# Autodesk Inventor assembly: Cangrejo-Sin-Reductores
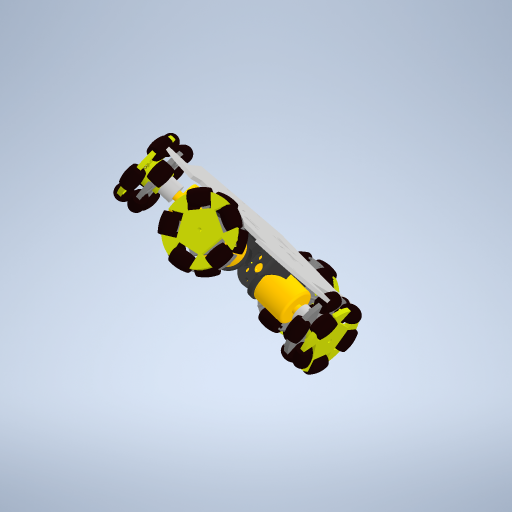
[picture p0: Inventor's stored thumbnail of the model, 512x512]
Saved by Autodesk Inventor 2024 (Build 280153000, 153)
## iProperties
Created: 2023-11-21
Part Number: Cangrejo-Sin-Reductores
Document SubType Name: Assembly
Designer: felip
Author: felip
## Documents named in this file (5)
- C:\Users\felip\Downloads\Gemelo Digital V2\Cangrejo-Sin-Reductores.iam
- C:\Users\felip\Downloads\Gemelo Digital V2\Motor-Soporte-Montaje.iam
- C:\Users\felip\Downloads\Gemelo Digital V2\OMNIWHEELV4.iam
- C:\Users\felip\Downloads\Gemelo Digital V2\Pseudo-SunGear.ipt
- C:\Users\felip\Downloads\Gemelo Digital V2\BaseV7.5.ipt
## Components (13 placed, 4 different names)
1. Motor-Soporte-Montaje:1 [sub-assembly] — Rotational:7, Rotational:22, Rotational:23
2. OMNIWHEELV4:1 [sub-assembly] — Rotational:14
3. Pseudo-SunGear:2 — Rotational:7, Rotational:17
4. Pseudo-SunGear:4 — Rotational:8, Rotational:14
5. Motor-Soporte-Montaje:2 [sub-assembly] — Rotational:8, Rotational:20, Rotational:21
6. OMNIWHEELV4:2 [sub-assembly] — Rotational:9
7. OMNIWHEELV4:4 [sub-assembly] — Rotational:17
8. Pseudo-SunGear:5 — Rotational:9
9. Motor-Soporte-Montaje:4 [sub-assembly] — Rotational:24, Rotational:25
10. OMNIWHEELV4:5 [sub-assembly]
11. Pseudo-SunGear:6
12. Motor-Soporte-Montaje:5 [sub-assembly] — Rotational:18, Rotational:19
13. BaseV7.5:1 — Rotational:18, Rotational:19, Rotational:20, Rotational:21, Rotational:22, Rotational:23, Rotational:24, Rotational:25
## Relationships (16: RevoluteJoint 16)
- [RevoluteJoint]: Pseudo-SunGear:5 ↔ Motor-Soporte-Montaje:4
- Rotational:7 [RevoluteJoint]: Motor-Soporte-Montaje:1 ↔ Pseudo-SunGear:2
- Rotational:8 [RevoluteJoint]: Pseudo-SunGear:4 ↔ Motor-Soporte-Montaje:2
- Rotational:9 [RevoluteJoint]: OMNIWHEELV4:2 ↔ Pseudo-SunGear:5
- [RevoluteJoint]: Pseudo-SunGear:6 ↔ Motor-Soporte-Montaje:5
- [RevoluteJoint]: OMNIWHEELV4:5 ↔ Pseudo-SunGear:6
- Rotational:14 [RevoluteJoint]: OMNIWHEELV4:1 ↔ Pseudo-SunGear:4
- Rotational:17 [RevoluteJoint]: Pseudo-SunGear:2 ↔ OMNIWHEELV4:4
- Rotational:18 [RevoluteJoint]: Motor-Soporte-Montaje:5 ↔ BaseV7.5:1
- Rotational:19 [RevoluteJoint]: Motor-Soporte-Montaje:5 ↔ BaseV7.5:1
- Rotational:20 [RevoluteJoint]: Motor-Soporte-Montaje:2 ↔ BaseV7.5:1
- Rotational:21 [RevoluteJoint]: Motor-Soporte-Montaje:2 ↔ BaseV7.5:1
- Rotational:22 [RevoluteJoint]: Motor-Soporte-Montaje:1 ↔ BaseV7.5:1
- Rotational:23 [RevoluteJoint]: Motor-Soporte-Montaje:1 ↔ BaseV7.5:1
- Rotational:24 [RevoluteJoint]: Motor-Soporte-Montaje:4 ↔ BaseV7.5:1
- Rotational:25 [RevoluteJoint]: Motor-Soporte-Montaje:4 ↔ BaseV7.5:1
## Named parameters: d10_d8 = 0 mm, d11_d9 = -164.051907 deg, d18_d10_d8 = 0 mm, d19_d11_d9 = -157.909117 deg, d20_d16 = 0 mm, d21_d17 = 19.220792 deg
